# Autodesk Inventor assembly: IRSensorMount
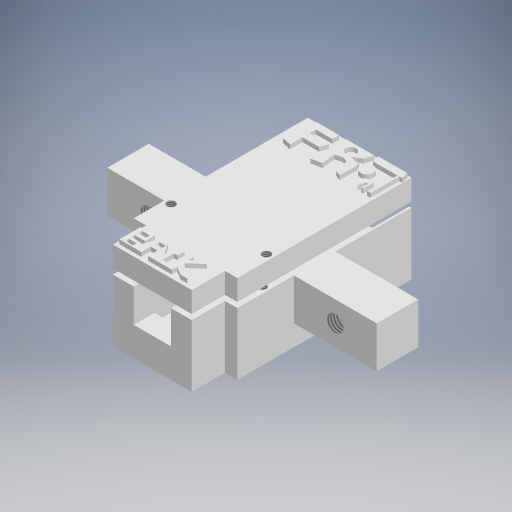
[picture p0: Inventor's stored thumbnail of the model, 512x512]
Saved by Autodesk Inventor 2023 (Build 270158000, 158)
## iProperties
Created: 2024-04-01
Part Number: IRSensorMount
Document SubType Name: Assembly
Designer: andrew
Author: andrew
## Documents named in this file (3)
- C:\Users\andre\Year4\EE579\Sem2\IRSensorMount.iam
- C:\Users\andre\Year4\EE579\Sem2\Base.ipt
- C:\Users\andre\Year4\EE579\Sem2\Head.ipt
## Components (2 placed, 2 different names)
1. Base:1 — Flush:1, Flush:2
2. Head:1 — Flush:1, Flush:2
## Relationships (2: Flush 2)
- Flush:1: Base:1 ↔ Head:1
- Flush:2: Base:1 ↔ Head:1
